# Autodesk Inventor assembly: Link Adapter Assembly
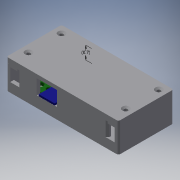
[picture p0: Inventor's stored thumbnail of the model, 180x180]
Saved by Autodesk Inventor 2017 (Build 210142000, 142)
## iProperties
Created: 2020-09-10
Part Number: Link Adapter Assembly
Document SubType Name: Assembly
Designer: Collin
Author: Collin
## Documents named in this file (4)
- C:\Users\Collin\Documents\Inventor\Link Adapter MtoM\Link Adapter Assembly.iam
- C:\Users\Collin\Documents\Inventor\Link Adapter MtoM\Link Adapter Top.ipt
- C:\Users\Collin\Documents\Inventor\Link Adapter MtoM\Link Adapter.ipt
- C:\Users\Collin\Documents\EAGLE\projects\GBA_SP_Link_Extender\untitled.brd.iam
## Components (3 placed, 3 different names)
1. Link Adapter Top:1 — Flush:1, Flush:2, Mate:1
2. Link Adapter:1 — Flush:1, Flush:2, Mate:1, Mate:2, Mate:3, Mate:4
3. untitled.brd:1 [sub-assembly] — Mate:2, Mate:3, Mate:4
## Relationships (6: Mate 4, Flush 2)
- Flush:1: Link Adapter Top:1 ↔ Link Adapter:1
- Flush:2: Link Adapter Top:1 ↔ Link Adapter:1
- Mate:1: Link Adapter Top:1 ↔ Link Adapter:1
- Mate:2: Link Adapter:1 ↔ untitled.brd:1
- Mate:3: Link Adapter:1 ↔ untitled.brd:1
- Mate:4: Link Adapter:1 ↔ untitled.brd:1
